# Autodesk Inventor assembly: tripleDiff
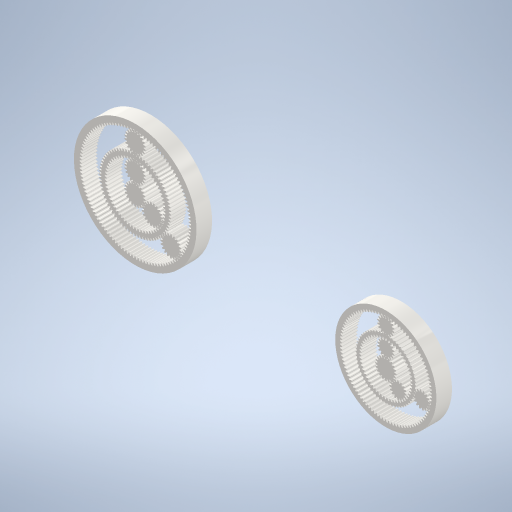
[picture p0: Inventor's stored thumbnail of the model, 512x512]
Saved by Autodesk Inventor 2023 (Build 270158000, 158)
## iProperties
Created: 2022-09-26
Part Number: tripleDiff
Document SubType Name: Assembly
Designer: deli
Author: deli
## Documents named in this file (9)
- C:\Users\deli\OneDrive - Eastside Preparatory School\FTC\8103-power-play\CAD\tripleDiff.iam
- C:\Users\deli\OneDrive - Eastside Preparatory School\FTC\8103-power-play\CAD\tripleDiff\Design Accelerator\Spur Gears4.iam
- C:\Users\deli\OneDrive - Eastside Preparatory School\FTC\8103-power-play\CAD\tripleDiff\Design Accelerator\Spur Gears6.iam
- C:\Users\deli\OneDrive - Eastside Preparatory School\FTC\8103-power-play\CAD\tripleDiff\Design Accelerator\Spur Gears11.iam
- C:\Users\deli\OneDrive - Eastside Preparatory School\FTC\8103-power-play\CAD\tripleDiff\Design Accelerator\Spur Gears12.iam
- C:\Users\deli\OneDrive - Eastside Preparatory School\FTC\8103-power-play\CAD\tripleDiff\Design Accelerator\Spur Gears14.iam
- C:\Users\deli\OneDrive - Eastside Preparatory School\FTC\8103-power-play\CAD\tripleDiff\Design Accelerator\Spur Gears15.iam
- C:\Users\deli\OneDrive - Eastside Preparatory School\FTC\8103-power-play\CAD\tripleDiff\Design Accelerator\Spur Gears18.iam
- C:\Users\deli\OneDrive - Eastside Preparatory School\FTC\8103-power-play\CAD\tripleDiff\Design Accelerator\Spur Gears20.iam
## Components (8 placed, 1 different names)
1. Spur Gears:1 [sub-assembly] — Mate:1, Flush:1
2. Spur Gears:2 [sub-assembly] — Mate:1, Flush:1, Mate:2, Flush:2, Flush:3
3. Spur Gears:3 [sub-assembly] — Mate:2, Flush:2, Mate:3, Flush:3
4. Spur Gears:4 [sub-assembly] — Mate:3
5. Spur Gears:5 [sub-assembly] — Flush:4, Mate:6
6. Spur Gears:6 [sub-assembly] — Flush:4, Mate:4, Flush:5, Flush:6, Mate:6
7. Spur Gears:7 [sub-assembly] — Mate:4, Flush:5, Mate:5
8. Spur Gears:8 [sub-assembly] — Mate:5, Flush:6
## Relationships (12: Mate 6, Flush 6)
- Mate:1: Spur Gears:1 ↔ Spur Gears:2
- Flush:1: Spur Gears:1 ↔ Spur Gears:2
- Mate:2: Spur Gears:2 ↔ Spur Gears:3
- Flush:2: Spur Gears:2 ↔ Spur Gears:3
- Mate:3: Spur Gears:3 ↔ Spur Gears:4
- Flush:3: Spur Gears:2 ↔ Spur Gears:3
- Flush:4: Spur Gears:5 ↔ Spur Gears:6
- Mate:4: Spur Gears:6 ↔ Spur Gears:7
- Flush:5: Spur Gears:6 ↔ Spur Gears:7
- Mate:5: Spur Gears:7 ↔ Spur Gears:8
- Flush:6: Spur Gears:6 ↔ Spur Gears:8
- Mate:6: Spur Gears:5 ↔ Spur Gears:6
